# Autodesk Inventor assembly: Drome(2)
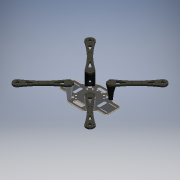
[picture p0: Inventor's stored thumbnail of the model, 180x180]
Saved by Autodesk Inventor 2018 (Build 220112000, 112)
## iProperties
Created: 2019-02-18
Part Number: Drome(2)
Document SubType Name: Assembly
Designer: anirudh
Author: anirudh
## Documents named in this file (4)
- C:\Users\anirudh\Documents\MARS Fund\Drone Stuff\dronePrototype2\Drome(2).iam
- C:\Users\anirudh\Documents\MARS Fund\Drone Stuff\dronePrototype2\ArmBracket(2).ipt
- C:\Users\anirudh\Documents\MARS Fund\Drone Stuff\dronePrototype2\FlameWheel_F450_Base_Bottom(2).ipt
- C:\Users\anirudh\Documents\MARS Fund\Drone Stuff\dronePrototype2\MotorLink(2).ipt
## Components (9 placed, 3 different names)
1. ArmBracket(2):1 — Flush:1, Mate:1, Mate:2, Mate:3, Symmetry:1, Mate:18, Mate:19, Mate:20, Mate:21, Mate:22
2. FlameWheel_F450_Base_Bottom(2):1 — Flush:1, Mate:1, Mate:2, Mate:3, Flush:2, Mate:4, Mate:5, Mate:6, Flush:3, Mate:7, Mate:8, Mate:9, Flush:4, Mate:10, Mate:11, Mate:12
3. MotorLink(2):1 — Flush:6, Mate:27, Mate:28, Mate:29, Mate:30
4. ArmBracket(2):2 — Flush:2, Mate:4, Mate:5, Mate:6, Flush:5, Mate:23, Mate:24, Mate:25, Mate:26
5. MotorLink(2):2 — Symmetry:1, Mate:18, Mate:19, Mate:20, Mate:21, Mate:22
6. ArmBracket(2):3 — Flush:3, Mate:7, Mate:8, Mate:9, Flush:6, Mate:27, Mate:28, Mate:29, Mate:30
7. MotorLink(2):3 — Mate:13, Mate:14, Mate:15, Mate:16, Mate:17
8. ArmBracket(2):4 — Flush:4, Mate:10, Mate:11, Mate:12, Mate:13, Mate:14, Mate:15, Mate:16, Mate:17
9. MotorLink(2):4 — Flush:5, Mate:23, Mate:24, Mate:25, Mate:26
## Relationships (37: Mate 30, Flush 6, Symmetry 1)
- Flush:1: ArmBracket(2):1 ↔ FlameWheel_F450_Base_Bottom(2):1
- Mate:1: ArmBracket(2):1 ↔ FlameWheel_F450_Base_Bottom(2):1
- Mate:2: ArmBracket(2):1 ↔ FlameWheel_F450_Base_Bottom(2):1
- Mate:3: ArmBracket(2):1 ↔ FlameWheel_F450_Base_Bottom(2):1
- Flush:2: FlameWheel_F450_Base_Bottom(2):1 ↔ ArmBracket(2):2
- Mate:4: FlameWheel_F450_Base_Bottom(2):1 ↔ ArmBracket(2):2
- Mate:5: FlameWheel_F450_Base_Bottom(2):1 ↔ ArmBracket(2):2
- Mate:6: FlameWheel_F450_Base_Bottom(2):1 ↔ ArmBracket(2):2
- Flush:3: FlameWheel_F450_Base_Bottom(2):1 ↔ ArmBracket(2):3
- Mate:7: FlameWheel_F450_Base_Bottom(2):1 ↔ ArmBracket(2):3
- Mate:8: FlameWheel_F450_Base_Bottom(2):1 ↔ ArmBracket(2):3
- Mate:9: FlameWheel_F450_Base_Bottom(2):1 ↔ ArmBracket(2):3
- Flush:4: FlameWheel_F450_Base_Bottom(2):1 ↔ ArmBracket(2):4
- Mate:10: FlameWheel_F450_Base_Bottom(2):1 ↔ ArmBracket(2):4
- Mate:11: FlameWheel_F450_Base_Bottom(2):1 ↔ ArmBracket(2):4
- Mate:12: FlameWheel_F450_Base_Bottom(2):1 ↔ ArmBracket(2):4
- Mate:13: MotorLink(2):3 ↔ ArmBracket(2):4
- Mate:14: MotorLink(2):3 ↔ ArmBracket(2):4
- Mate:15: MotorLink(2):3 ↔ ArmBracket(2):4
- Mate:16: MotorLink(2):3 ↔ ArmBracket(2):4
- Mate:17: MotorLink(2):3 ↔ ArmBracket(2):4
- Symmetry:1: ArmBracket(2):1 ↔ MotorLink(2):2
- Mate:18: ArmBracket(2):1 ↔ MotorLink(2):2
- Mate:19: ArmBracket(2):1 ↔ MotorLink(2):2
- Mate:20: ArmBracket(2):1 ↔ MotorLink(2):2
- Mate:21: ArmBracket(2):1 ↔ MotorLink(2):2
- Mate:22: ArmBracket(2):1 ↔ MotorLink(2):2
- Flush:5: ArmBracket(2):2 ↔ MotorLink(2):4
- Mate:23: ArmBracket(2):2 ↔ MotorLink(2):4
- Mate:24: ArmBracket(2):2 ↔ MotorLink(2):4
- Mate:25: ArmBracket(2):2 ↔ MotorLink(2):4
- Mate:26: ArmBracket(2):2 ↔ MotorLink(2):4
- Flush:6: MotorLink(2):1 ↔ ArmBracket(2):3
- Mate:27: MotorLink(2):1 ↔ ArmBracket(2):3
- Mate:28: MotorLink(2):1 ↔ ArmBracket(2):3
- Mate:29: MotorLink(2):1 ↔ ArmBracket(2):3
- Mate:30: MotorLink(2):1 ↔ ArmBracket(2):3
